# Autodesk Inventor assembly: BoronProbe_2026_non-rotating_1
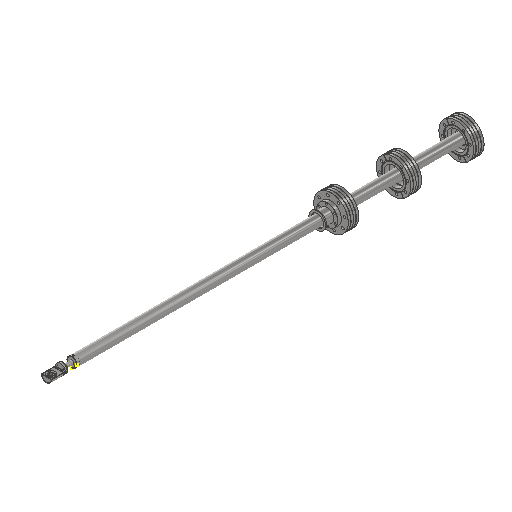
[picture p0: Inventor's stored thumbnail of the model, 512x512]
Saved by Autodesk Inventor 2026.2 (Build 302298000, 298)
## iProperties
Created: 2026-05-08
Part Number: BoronProbe_2026_non-rotating_1
Document SubType Name: Assembly
Designer: zetsu
ProbePos: 413.000 mm
Author: zetsu
## Documents named in this file (12)
- D:\repos\PIHTI\BoronProbe_2026\BoronProbe_2026_non-rotating_1.iam
- D:\repos\PIHTI\BoronProbe_2026\parts\C25K22A4CU.iam
- D:\repos\PIHTI\BoronProbe_2026\parts\ICF114-through.ipt
- D:\repos\PIHTI\BoronProbe_2026\parts\ICF70_to_KF40.ipt
- D:\repos\PIHTI\BoronProbe_2026\parts\B_probe_bearing.ipt
- D:\repos\PIHTI\BoronProbe_2026\parts\ICF_114-70_bearing.ipt
- D:\repos\PIHTI\BoronProbe_2026\parts\B_pipe_flange_spacer_5.ipt
- D:\repos\PIHTI\BoronProbe_2026\parts\M4×12-VentedHexBolt.ipt
- D:\repos\PIHTI\Plasma Vessel_2026\contents\ICF_114-70.ipt
- D:\repos\PIHTI\BoronProbe_2026\SampleHolder_1.iam
- D:\repos\PIHTI\BoronProbe_2026\parts\B_probe_pipe_5_for-non-rotating_1.ipt
- D:\repos\PIHTI\BoronProbe_2026\parts\M2-4_screw.ipt
## Components (19 placed, 11 different names)
1. C25K22A4CU:1 [sub-assembly]
2. B_probe_pipe_5_for-non-rotating_1:1 — メイト:158, メイト:159, メイト:160, メイト:167, メイト:168, 挿入:1, 挿入:2, 挿入:3, 挿入:4
3. ICF_114-70:1 — メイト:121, メイト:122, メイト:137, メイト:158, フラッシュ:7
4. ICF114-through:1 — メイト:121, メイト:122, メイト:123, メイト:124, メイト:137, フラッシュ:5, フラッシュ:6
5. ICF114-through:2 — メイト:123, メイト:124, メイト:125, メイト:126, メイト:127, メイト:129
6. ICF114-through:3 — メイト:125, メイト:126, メイト:127, メイト:128, フラッシュ:5
7. ICF114-through:4 — メイト:128, メイト:129, メイト:130, メイト:131, メイト:132, 角度:1
8. ICF_114-70_bearing:2 — メイト:130, メイト:131, メイト:132, メイト:133, メイト:134, メイト:138, メイト:139, フラッシュ:6, メイト:151
9. ICF70_to_KF40:1 — メイト:133, メイト:134, 角度:1
10. B_probe_bearing:2 — メイト:138, メイト:139, メイト:151, メイト:161, メイト:162, メイト:163, メイト:164, メイト:165, メイト:166
11. B_pipe_flange_spacer_5:1 — メイト:159, メイト:160, フラッシュ:7
12. M4×12-VentedHexBolt:1 — メイト:161, メイト:162
13. M4×12-VentedHexBolt:2 — メイト:163, メイト:164
14. M4×12-VentedHexBolt:3 — メイト:165, メイト:166
15. SampleHolder_1:1 [sub-assembly] — メイト:167, メイト:168
16. M2-4_screw:1 — 挿入:1
17. M2-4_screw:2 — 挿入:2
18. M2-4_screw:3 — 挿入:3
19. M2-4_screw:4 — 挿入:4
## Relationships (37: Mate 29, Insert 4, Flush 3, Angle 1)
- メイト:121 [Mate]: ICF_114-70:1 ↔ ICF114-through:1
- メイト:122 [Mate]: ICF_114-70:1 ↔ ICF114-through:1
- メイト:123 [Mate]: ICF114-through:1 ↔ ICF114-through:2
- メイト:124 [Mate]: ICF114-through:1 ↔ ICF114-through:2
- メイト:125 [Mate]: ICF114-through:2 ↔ ICF114-through:3
- メイト:126 [Mate]: ICF114-through:2 ↔ ICF114-through:3
- メイト:127 [Mate]: ICF114-through:2 ↔ ICF114-through:3
- メイト:128 [Mate]: ICF114-through:3 ↔ ICF114-through:4
- メイト:129 [Mate]: ICF114-through:2 ↔ ICF114-through:4
- メイト:130 [Mate]: ICF114-through:4 ↔ ICF_114-70_bearing:2
- メイト:131 [Mate]: ICF114-through:4 ↔ ICF_114-70_bearing:2
- メイト:132 [Mate]: ICF114-through:4 ↔ ICF_114-70_bearing:2
- メイト:133 [Mate]: ICF_114-70_bearing:2 ↔ ICF70_to_KF40:1
- メイト:134 [Mate]: ICF_114-70_bearing:2 ↔ ICF70_to_KF40:1
- 角度:1 [Angle] (0 deg): ICF114-through:4 ↔ ICF70_to_KF40:1
- メイト:137 [Mate]: ICF_114-70:1 ↔ ICF114-through:1
- メイト:138 [Mate]: ICF_114-70_bearing:2 ↔ B_probe_bearing:2
- メイト:139 [Mate]: ICF_114-70_bearing:2 ↔ B_probe_bearing:2
- フラッシュ:5 [Flush] (206.5 mm): ICF114-through:1 ↔ ICF114-through:3
- フラッシュ:6 [Flush] (413 mm): ICF114-through:1 ↔ ICF_114-70_bearing:2
- メイト:151 [Mate]: ICF_114-70_bearing:2 ↔ B_probe_bearing:2
- メイト:158 [Mate]: B_probe_pipe_5_for-non-rotating_1:1 ↔ ICF_114-70:1
- メイト:159 [Mate]: B_probe_pipe_5_for-non-rotating_1:1 ↔ B_pipe_flange_spacer_5:1
- メイト:160 [Mate]: B_probe_pipe_5_for-non-rotating_1:1 ↔ B_pipe_flange_spacer_5:1
- フラッシュ:7 [Flush]: ICF_114-70:1 ↔ B_pipe_flange_spacer_5:1
- メイト:161 [Mate]: B_probe_bearing:2 ↔ M4×12-VentedHexBolt:1
- メイト:162 [Mate]: B_probe_bearing:2 ↔ M4×12-VentedHexBolt:1
- メイト:163 [Mate]: B_probe_bearing:2 ↔ M4×12-VentedHexBolt:2
- メイト:164 [Mate]: B_probe_bearing:2 ↔ M4×12-VentedHexBolt:2
- メイト:165 [Mate]: B_probe_bearing:2 ↔ M4×12-VentedHexBolt:3
- メイト:166 [Mate]: B_probe_bearing:2 ↔ M4×12-VentedHexBolt:3
- メイト:167 [Mate]: B_probe_pipe_5_for-non-rotating_1:1 ↔ SampleHolder_1:1
- メイト:168 [Mate]: B_probe_pipe_5_for-non-rotating_1:1 ↔ SampleHolder_1:1
- 挿入:1 [Insert]: B_probe_pipe_5_for-non-rotating_1:1 ↔ M2-4_screw:1
- 挿入:2 [Insert]: B_probe_pipe_5_for-non-rotating_1:1 ↔ M2-4_screw:2
- 挿入:3 [Insert]: B_probe_pipe_5_for-non-rotating_1:1 ↔ M2-4_screw:3
- 挿入:4 [Insert]: B_probe_pipe_5_for-non-rotating_1:1 ↔ M2-4_screw:4
## Named parameters: ProbePos = 413 mm, ProbePos_Max = 413 mm, ProbePos_Min = 760 mm
